# Autodesk Inventor assembly: sphericalFourBar
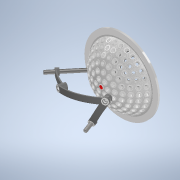
[picture p0: Inventor's stored thumbnail of the model, 180x180]
Saved by Autodesk Inventor 2020.1 (Build 241239000, 239)
## iProperties
Created: 2019-08-08
Part Number: sphericalFourBar
Document SubType Name: Assembly
Designer: sshel
Author: sshel
## Documents named in this file (6)
- C:\Users\sshel\Downloads\Compressed\spherical-mechanisms-puzzle-1.snapshot.2\spherical four bar\New folder\sphericalFourBar.iam
- C:\Users\sshel\Downloads\Compressed\spherical-mechanisms-puzzle-1.snapshot.2\spherical four bar\New folder\Spherical Base.ipt
- C:\Users\sshel\Downloads\Compressed\spherical-mechanisms-puzzle-1.snapshot.2\spherical four bar\New folder\Inp_Ang20_levelLow.ipt
- C:\Users\sshel\Downloads\Compressed\spherical-mechanisms-puzzle-1.snapshot.2\spherical four bar\New folder\Out_Ang30_levelLow.ipt
- C:\Users\sshel\Downloads\Compressed\spherical-mechanisms-puzzle-1.snapshot.2\spherical four bar\New folder\Cplr_Ang45_levelHigh.ipt
- C:\Users\sshel\Downloads\Compressed\spherical-mechanisms-puzzle-1.snapshot.2\spherical four bar\New folder\Shaft.ipt
## Components (6 placed, 5 different names)
1. Spherical Base:1 — ShaftInpPlane, ShaftInpAxis, ShaftOutPlane, ShaftOutAxis, SphInp, FPInp, SphOut, FPOut
2. Shaft:1 — ShaftInpPlane, ShaftInpAxis
3. Shaft:2 — ShaftOutPlane, ShaftOutAxis
4. Inp_Ang20_levelLow:1 — SphInp, FPInp, MPInp
5. Out_Ang30_levelLow:1 — SphOut, FPOut, MPOut
6. Cplr_Ang45_levelHigh:1 — MPInp, MPOut
## Relationships (10: Mate 10)
- ShaftInpPlane [Mate]: Spherical Base:1 ↔ Shaft:1
- ShaftInpAxis [Mate]: Spherical Base:1 ↔ Shaft:1
- ShaftOutPlane [Mate]: Spherical Base:1 ↔ Shaft:2
- ShaftOutAxis [Mate]: Spherical Base:1 ↔ Shaft:2
- SphInp [Mate]: Spherical Base:1 ↔ Inp_Ang20_levelLow:1
- FPInp [Mate]: Spherical Base:1 ↔ Inp_Ang20_levelLow:1
- SphOut [Mate]: Spherical Base:1 ↔ Out_Ang30_levelLow:1
- FPOut [Mate]: Spherical Base:1 ↔ Out_Ang30_levelLow:1
- MPInp [Mate]: Inp_Ang20_levelLow:1 ↔ Cplr_Ang45_levelHigh:1
- MPOut [Mate]: Out_Ang30_levelLow:1 ↔ Cplr_Ang45_levelHigh:1
